# Autodesk Inventor assembly: SC-0-01-ICE Assembly
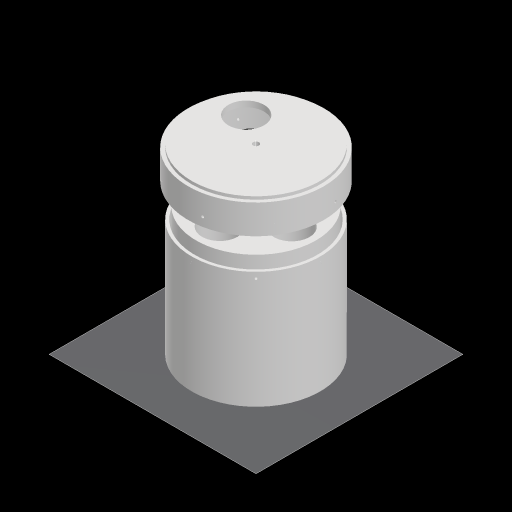
[picture p0: Inventor's stored thumbnail of the model, 512x512]
Saved by Autodesk Inventor 2023 (Build 270158000, 158)
## iProperties
Created: 2023-12-31
Part Number: SC-0-01-ICE Assembly
Document SubType Name: Assembly
Designer: annah
Author: annah
## Documents named in this file (4)
- C:\Users\annah\Documents\GitHub\BehrendURCMechanical\CAD\Science\SC-0-01-ICE Assembly.iam
- C:\Users\annah\Documents\GitHub\BehrendURCMechanical\CAD\Science\SC-1-01-Housing for Ice Holder.ipt
- C:\Users\annah\Documents\GitHub\BehrendURCMechanical\CAD\Science\SC-1-01-Housing lid.ipt
- C:\Users\annah\Documents\GitHub\BehrendURCMechanical\CAD\Science\SC-1-01-Ice Core Holder.ipt
## Components (3 placed, 3 different names)
1. SC-1-01-Housing lid:1 — Mate:5
2. SC-1-01-Housing for Ice Holder:1 — Mate:1, Mate:2, Rotation:1, Mate:3, Mate:4, Mate:5
3. SC-1-01-Ice Core Holder:1 — Mate:3, Mate:4
## Relationships (6: Mate 5, RelateRotation 1)
- Mate:1: SC-1-01-Housing for Ice Holder:1
- Mate:2: SC-1-01-Housing for Ice Holder:1
- Rotation:1 [RelateRotation] (1 ul): SC-1-01-Housing for Ice Holder:1
- Mate:3: SC-1-01-Housing for Ice Holder:1 ↔ SC-1-01-Ice Core Holder:1
- Mate:4: SC-1-01-Housing for Ice Holder:1 ↔ SC-1-01-Ice Core Holder:1
- Mate:5: SC-1-01-Housing lid:1 ↔ SC-1-01-Housing for Ice Holder:1
